# Autodesk Inventor assembly: oxidiser tank
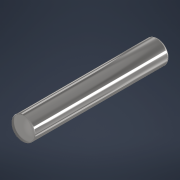
[picture p0: Inventor's stored thumbnail of the model, 180x180]
Saved by Autodesk Inventor 2021 (Build 250183000, 183)
## iProperties
Created: 2020-12-02
Part Number: oxidiser tank
Document SubType Name: Assembly
Designer: henry
Author: henry
## Documents named in this file (3)
- C:\Users\henry\Desktop\rocket\cad\tanks\oxidiser tank.iam
- C:\Users\henry\Desktop\rocket\cad\tanks\oxidiser tank wall.ipt
- C:\Users\henry\Desktop\rocket\cad\tanks\tank endcap.ipt
## Components (3 placed, 2 different names)
1. oxidiser tank wall:1 — Mate:1, Mate:2
2. tank endcap:1 — Mate:2
3. tank endcap:2 — Mate:1
## Relationships (2: Mate 2)
- Mate:1: oxidiser tank wall:1 ↔ tank endcap:2
- Mate:2: oxidiser tank wall:1 ↔ tank endcap:1
